# Autodesk Inventor assembly: 42146-08
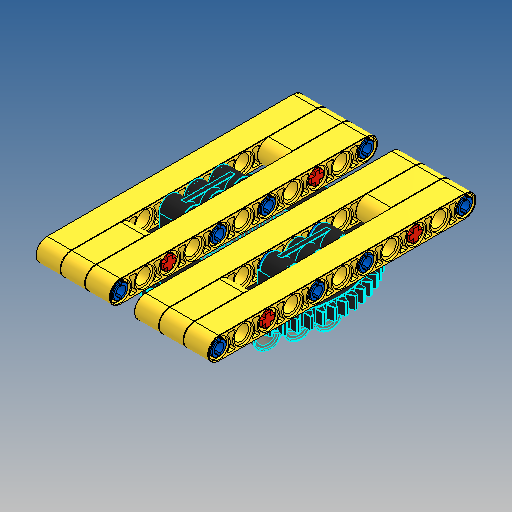
[picture p0: Inventor's stored thumbnail of the model, 512x512]
Saved by Autodesk Inventor 2025.1 (Build 291241000, 241)
## iProperties
Created: 2024-11-16
Part Number: 42146-08
Material: Generisch
Document SubType Name: Assembly
Designer: hp.muther
Author: hp.muther
## Documents named in this file (6)
- D:\Inventor\Projekte\Muther\LEGO Technic\LEGO Technik - Raupenkran LR 13000 (42146)\42146-08.iam
- D:\Inventor\Projekte\Muther\LEGO Technic\LEGO Pieces\Lochbalken\32525-Yellow.ipt
- D:\Inventor\Projekte\Muther\LEGO Technic\LEGO Pieces\Pin's\6558-Blue.ipt
- D:\Inventor\Projekte\Muther\LEGO Technic\LEGO Pieces\Pin's\11214-Red.ipt
- D:\Inventor\Projekte\Muther\LEGO Technic\LEGO Pieces\Lochbalken\32523-Yellow.ipt
- D:\Inventor\Projekte\Muther\LEGO Technic\LEGO Pieces\Zahnrad\48452cx1-DkBluishGray.iam
## Components (21 placed, 5 different names)
1. 32525-Yellow:1 — Winkel:1, Einfügen:1, Einfügen:2, Einfügen:3, Einfügen:4, Einfügen:7, Einfügen:8, Passend:1, Passend:2, Einfügen:10
2. 32525-Yellow:2 — Passend:3, Einfügen:9
3. 6558-Blue:1 — Einfügen:3
4. 6558-Blue:2 — Einfügen:4
5. 6558-Blue:3 — Einfügen:1, Passend:3
6. 6558-Blue:4 — Einfügen:2, Passend:4
7. 11214-Red:1 — Einfügen:5, Passend:2
8. 11214-Red:2 — Einfügen:6, Passend:1
9. 32523-Yellow:1 — Einfügen:6, Einfügen:8
10. 32523-Yellow:2 — Einfügen:5, Einfügen:7, Einfügen:9
11. 48452cx1-DkBluishGray:1 [sub-assembly] — Einfügen:10, Passend:4, Einfügen:20, Passend:8, Winkel:1
12. 32525-Yellow:3 — Einfügen:20
13. 32525-Yellow:4
14. 6558-Blue:5
15. 6558-Blue:6
16. 6558-Blue:7
17. 6558-Blue:8 — Passend:8
18. 11214-Red:3
19. 11214-Red:4
20. 32523-Yellow:3
21. 32523-Yellow:4
## Relationships (29: Insert 20, Mate 8, Angle 1)
- Winkel:1 [Angle] (0 deg): 32525-Yellow:1 ↔ 48452cx1-DkBluishGray:1
- Einfügen:1 [Insert]: 32525-Yellow:1 ↔ 6558-Blue:3
- Einfügen:2 [Insert]: 32525-Yellow:1 ↔ 6558-Blue:4
- Einfügen:3 [Insert]: 32525-Yellow:1 ↔ 6558-Blue:1
- Einfügen:4 [Insert]: 32525-Yellow:1 ↔ 6558-Blue:2
- Einfügen:5 [Insert]: 11214-Red:1 ↔ 32523-Yellow:2
- Einfügen:6 [Insert]: 11214-Red:2 ↔ 32523-Yellow:1
- Einfügen:7 [Insert]: 32525-Yellow:1 ↔ 32523-Yellow:2
- Einfügen:8 [Insert]: 32525-Yellow:1 ↔ 32523-Yellow:1
- Passend:1 [Mate]: 32525-Yellow:1 ↔ 11214-Red:2
- Passend:2 [Mate]: 32525-Yellow:1 ↔ 11214-Red:1
- Passend:3 [Mate]: 32525-Yellow:2 ↔ 6558-Blue:3
- Einfügen:9 [Insert]: 32525-Yellow:2 ↔ 32523-Yellow:2
- Einfügen:10 [Insert]: 32525-Yellow:1 ↔ 48452cx1-DkBluishGray:1
- Passend:4 [Mate]: 6558-Blue:4 ↔ 48452cx1-DkBluishGray:1
- [Insert]: 32525-Yellow:3 ↔ 6558-Blue:7
- [Insert]: 32525-Yellow:3 ↔ 6558-Blue:8
- [Insert]: 32525-Yellow:3 ↔ 6558-Blue:5
- [Insert]: 32525-Yellow:3 ↔ 6558-Blue:6
- [Insert]: 11214-Red:3 ↔ 32523-Yellow:4
- [Insert]: 11214-Red:4 ↔ 32523-Yellow:3
- [Insert]: 32525-Yellow:3 ↔ 32523-Yellow:4
- [Insert]: 32525-Yellow:3 ↔ 32523-Yellow:3
- [Mate]: 32525-Yellow:3 ↔ 11214-Red:4
- [Mate]: 32525-Yellow:3 ↔ 11214-Red:3
- [Mate]: 32525-Yellow:4 ↔ 6558-Blue:7
- [Insert]: 32525-Yellow:4 ↔ 32523-Yellow:4
- Einfügen:20 [Insert]: 48452cx1-DkBluishGray:1 ↔ 32525-Yellow:3
- Passend:8 [Mate]: 48452cx1-DkBluishGray:1 ↔ 6558-Blue:8
## Named parameters: d14_d8 = 0 mm, d15_d9 = 0 mm, d16_d10 = 0 mm, d17_d11 = 0 mm, d18_d1 = 0 mm, d19_d2 = 0 mm, d20_d3 = 0 mm, d21_d4 = 0 mm, d22_d5 = 0 mm, d23_d6 = 0 mm, d24_d7 = 0 mm, d25_d0 = 0 mm
